# Autodesk Inventor assembly: Assembly1
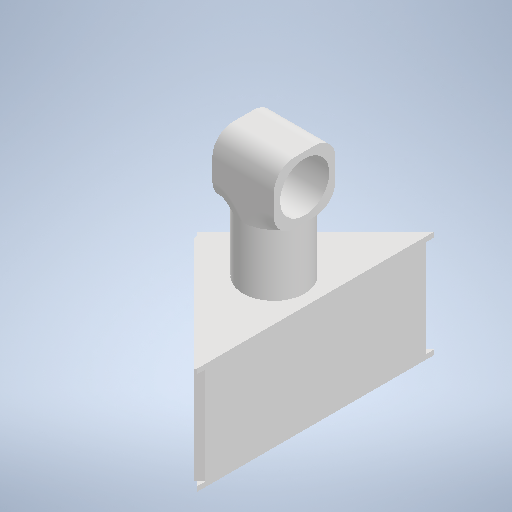
[picture p0: Inventor's stored thumbnail of the model, 512x512]
Saved by Autodesk Inventor 2025.2 (Build 292293000, 293)
## iProperties
Created: 2025-07-25
Part Number: Assembly1
Document SubType Name: Assembly
Designer: arbaz
Author: arbaz
## Documents named in this file (3)
- C:\Users\arbaz\OneDrive\Documents\Ritesh\Assembly1.iam
- C:\Users\arbaz\OneDrive\Documents\Ritesh\SolarPannelMounting.ipt
- C:\Users\arbaz\OneDrive\Documents\Ritesh\Holder.ipt
## Components (2 placed, 2 different names)
1. SolarPannelMounting:1 — Flush:1
2. Holder:1 — Flush:1
## Relationships (1: Flush 1)
- Flush:1: SolarPannelMounting:1 ↔ Holder:1
